# Autodesk Inventor assembly: Actuator
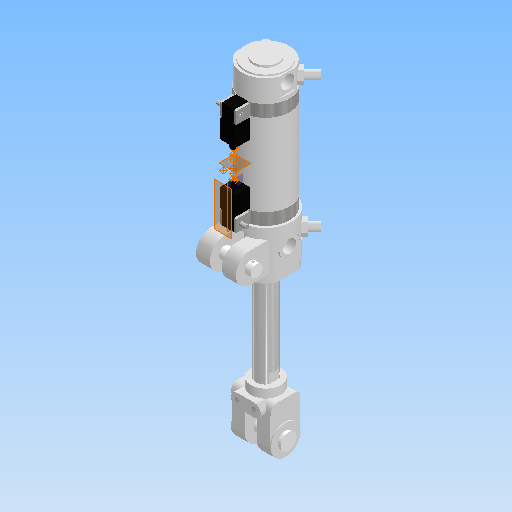
[picture p0: Inventor's stored thumbnail of the model, 512x512]
Saved by Autodesk Inventor 2020.1 (Build 241239000, 239)
## iProperties
Created: 2019-08-27
Part Number: Actuator
Document SubType Name: Assembly
Designer: thom_tremblay
Author: thom_tremblay
## Documents named in this file (3)
- C:\Users\thom_tremblay\Desktop\Inventor ACP Data\Assemblies\Actuator.iam
- C:\Users\thom_tremblay\Desktop\Inventor ACP Data\Assemblies\PH-000-001.iam
- C:\Users\thom_tremblay\Desktop\Inventor ACP Data\Assemblies\PH-000-002.iam
## Components (2 placed, 2 different names)
1. PH-000-002:1 [sub-assembly]
2. PH-000-001:1 [sub-assembly]
## Relationships (1: Mate 1)
- [Mate]: PH-000-002:1 ↔ PH-000-001:1
